# Autodesk Inventor assembly: assembly
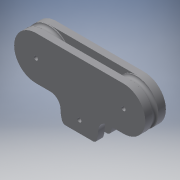
[picture p0: Inventor's stored thumbnail of the model, 180x180]
Saved by Autodesk Inventor 2016 (Build 200138000, 138)
## iProperties
Created: 2019-02-22
Part Number: assembly
Document SubType Name: Assembly
Designer: reesem783
Author: reesem783
## Documents named in this file (4)
- H:\Github\Zipline\Inventor\assembly.iam
- H:\Github\Zipline\Inventor\wheel.ipt
- H:\Github\Zipline\Inventor\casing.ipt
- H:\Github\Zipline\Inventor\bearing.ipt
## Components (6 placed, 3 different names)
1. wheel:1 — Mate:1, Mate:2, Insert:2, Mate:5
2. wheel:2 — Mate:3, Mate:4, Insert:1, Mate:6
3. casing:1 — Mate:1, Mate:2, Mate:3, Mate:4, Mate:7
4. casing:2 — Mate:5, Mate:6, Mate:7
5. bearing:1 — Insert:1
6. bearing:2 — Insert:2
## Relationships (9: Mate 7, Insert 2)
- Mate:1: wheel:1 ↔ casing:1
- Mate:2: wheel:1 ↔ casing:1
- Mate:3: wheel:2 ↔ casing:1
- Mate:4: wheel:2 ↔ casing:1
- Insert:1: wheel:2 ↔ bearing:1
- Insert:2: wheel:1 ↔ bearing:2
- Mate:5: wheel:1 ↔ casing:2
- Mate:6: wheel:2 ↔ casing:2
- Mate:7: casing:1 ↔ casing:2
